# Autodesk Inventor assembly: mould_casing_testfit
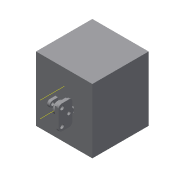
[picture p0: Inventor's stored thumbnail of the model, 180x180]
Saved by Autodesk Inventor 2017 (Build 210142000, 142)
## iProperties
Created: 2018-06-07
Part Number: mould_casing_testfit
Document SubType Name: Assembly
Designer: Nic
Author: Nic
## Documents named in this file (4)
- C:\Users\Nic\Documents\Antenna\mould_casing_testfit.iam
- C:\Users\Nic\Documents\Antenna\mould_casing_base_v2.ipt
- C:\Users\Nic\Documents\Antenna\middle_segment_v2.ipt
- C:\Users\Nic\Documents\Antenna\mould_casing_top_v2.ipt
## Components (3 placed, 3 different names)
1. mould_casing_base_v2:1 — Mate:1, Mate:2, Mate:3, Insert:1, Insert:2
2. middle_segment_v2:1 — Mate:1, Mate:2, Mate:3
3. mould_casing_top_v2:1 — Insert:1, Insert:2
## Relationships (5: Mate 3, Insert 2)
- Mate:1 (0.2 mm): mould_casing_base_v2:1 ↔ middle_segment_v2:1
- Mate:2 (0.2 mm): mould_casing_base_v2:1 ↔ middle_segment_v2:1
- Mate:3 (0.2 mm): mould_casing_base_v2:1 ↔ middle_segment_v2:1
- Insert:1: mould_casing_base_v2:1 ↔ mould_casing_top_v2:1
- Insert:2: mould_casing_base_v2:1 ↔ mould_casing_top_v2:1
